# Autodesk Inventor assembly: Test_Assembly
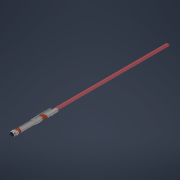
[picture p0: Inventor's stored thumbnail of the model, 180x180]
Saved by Autodesk Inventor 2022 (Build 260153000, 153)
## iProperties
Created: 2024-05-08
Part Number: Test_Assembly
Document SubType Name: Assembly
Designer: jo_ki
Author: jo_ki
## Documents named in this file (16)
- C:\LocalRepos\Lightsaber Git\CAD\LightSaber_Inventor_Project\Assemblies\Blade_Assembly.iam
- C:\LocalRepos\Lightsaber Git\CAD\LightSaber_Inventor_Project\Parts\Blade_Guard.ipt
- C:\LocalRepos\Lightsaber Git\CAD\LightSaber_Inventor_Project\Parts\Saber_Body.ipt
- C:\LocalRepos\Lightsaber Git\CAD\LightSaber_Inventor_Project\Parts\Emitter_Barrel.ipt
- C:\LocalRepos\Lightsaber Git\CAD\LightSaber_Inventor_Project\Parts\Radiator.ipt
- C:\LocalRepos\Lightsaber Git\CAD\LightSaber_Inventor_Project\Parts\Blade.ipt
- C:\LocalRepos\Lightsaber Git\CAD\LightSaber_Inventor_Project\Parts\Endcap.ipt
- C:\LocalRepos\Lightsaber Git\CAD\LightSaber_Inventor_Project\Parts\Decal_Ring_Tripple.ipt
- C:\Users\jo_ki\OneDrive\Dokumente\Inventor\Content Center Files\R2022\en-US\ISO 4762(2)\ISO 4762 - M2.5 x 5ISO.ipt
- C:\Users\jo_ki\OneDrive\Dokumente\Inventor\Content Center Files\R2022\en-US\ISO 4762(2)\ISO 4762 - M2.5 x 4ISO.ipt
- C:\LocalRepos\Lightsaber Git\CAD\LightSaber_Inventor_Project\Parts\Blade_Holder.ipt
- C:\Users\jo_ki\OneDrive\Dokumente\Inventor\Content Center Files\R2022\en-US\DIN 913\DIN 913 - M2.5 x 6.ipt
- C:\Users\jo_ki\OneDrive\Dokumente\Inventor\Content Center Files\R2022\en-US\ISO 4762(2)\ISO 4762 - M2.5 x 10ISO.ipt
- C:\LocalRepos\Lightsaber Git\CAD\LightSaber_Inventor_Project\Assemblies\Electronics_Assembly.iam
- C:\LocalRepos\Lightsaber Git\CAD\LightSaber_Inventor_Project\Parts\Radiator_Disc.ipt
- C:\LocalRepos\Lightsaber Git\CAD\LightSaber_Inventor_Project\Assemblies\Switch_Assembly.iam
## Components (30 placed, 15 different names)
1. Test_Blade_Guard:1 — Mate:1, Mate:52, Insert:2
2. Test_Body:1 — Mate:1, Mate:2, Mate:6, Angle:1, Mate:9, Mate:18, Mate:19, Mate:24, Mate:25, Mate:29, Mate:30, Mate:31, Mate:32, Mate:50, Mate:58, Mate:59, Mate:62, Mate:63, Mate:66, Mate:67, Mate:68, Flush:9, Mate:94
3. Test_Radiator:1 — Mate:9, Mate:50, Mate:51, Mate:54, Mate:71, Mate:72, Mate:73, Mate:74, Mate:75, Mate:76, Mate:77, Mate:78, Mate:79, Mate:80, Mate:81, Mate:82, Mate:83, Mate:84, Mate:85, Mate:86, Mate:89
4. Emitter_Barrel:1 — Mate:2, Mate:51, Mate:52, Mate:56, Mate:57, Mate:60, Mate:61, Insert:3, Insert:4
5. Blade:1 — Mate:19, Flush:1
6. Test_Endcap:1 — Mate:18, Mate:88
7. Test_Decal_Ring_Tripple:1 — Mate:24, Insert:1
8. Test_Decal_Ring_Tripple:2 — Mate:25, Mate:35, Mate:39, Mate:40
9. Test_Blade_Holder:1 — Mate:54, Flush:1
10. Electronics_Assembly:1 [sub-assembly] — Mate:68, Mate:88, Mate:89, Mate:94
11. Test_Radiator_Disc:1 — Mate:74, Mate:79, Flush:2
12. Test_Radiator_Disc:2 — Mate:75, Mate:84, Flush:7, Flush:8
13. Test_Radiator_Disc:3 — Mate:76, Mate:81, Flush:3, Flush:4
14. Test_Radiator_Disc:4 — Mate:77, Mate:82, Flush:4, Flush:5
15. Test_Radiator_Disc:5 — Mate:78, Mate:80, Flush:2, Flush:3
16. Test_Radiator_Disc:6 — Mate:73, Mate:83, Flush:5, Flush:6, Flush:9
17. Test_Radiator_Disc:7 — Mate:72, Flush:6, Flush:7, Mate:86
18. Test_Radiator_Disc:8 — Mate:71, Mate:85, Flush:8
19. Test_Switch_Assembly:1 [sub-assembly]
20. ISO 4762 M2.5 x 5:1 — Mate:29, Mate:30
21. ISO 4762 M2.5 x 5:2 — Mate:31, Mate:32
22. ISO 4762 M2.5 x 4:1 — Mate:39, Mate:40, Mate:67
23. ISO 4762 M2.5 x 4:2 — Insert:1, Mate:66
24. DIN 913 M2.5 x 6:1 — Mate:56, Mate:58
25. DIN 913 M2.5 x 6:2 — Mate:57, Mate:59
26. DIN 913 M2.5 x 6:3 — Mate:60, Mate:63
27. DIN 913 M2.5 x 6:4 — Mate:61, Mate:62
28. ISO 4762 M2.5 x 10:1 — Insert:2
29. ISO 4762 M2.5 x 5:3 — Insert:3
30. ISO 4762 M2.5 x 5:4 — Insert:4
## Relationships (65: Mate 51, Flush 9, Insert 4, Angle 1)
- Mate:1: Test_Blade_Guard:1 ↔ Test_Body:1
- Mate:2: Test_Body:1 ↔ Emitter_Barrel:1
- Mate:6: Test_Body:1
- Angle:1 (0 deg): Test_Body:1
- Mate:9: Test_Body:1 ↔ Test_Radiator:1
- Mate:18: Test_Body:1 ↔ Test_Endcap:1
- Mate:19: Test_Body:1 ↔ Blade:1
- Mate:24: Test_Body:1 ↔ Test_Decal_Ring_Tripple:1
- Mate:25: Test_Body:1 ↔ Test_Decal_Ring_Tripple:2
- Mate:29: Test_Body:1 ↔ ISO 4762 M2.5 x 5:1
- Mate:30: Test_Body:1 ↔ ISO 4762 M2.5 x 5:1
- Mate:31: Test_Body:1 ↔ ISO 4762 M2.5 x 5:2
- Mate:32: Test_Body:1 ↔ ISO 4762 M2.5 x 5:2
- Mate:35: Test_Decal_Ring_Tripple:2
- Mate:37
- Mate:38
- Mate:39: Test_Decal_Ring_Tripple:2 ↔ ISO 4762 M2.5 x 4:1
- Mate:40: Test_Decal_Ring_Tripple:2 ↔ ISO 4762 M2.5 x 4:1
- Insert:1: Test_Decal_Ring_Tripple:1 ↔ ISO 4762 M2.5 x 4:2
- Mate:50: Test_Body:1 ↔ Test_Radiator:1
- Mate:51: Test_Radiator:1 ↔ Emitter_Barrel:1
- Mate:52: Test_Blade_Guard:1 ↔ Emitter_Barrel:1
- Mate:54: Test_Radiator:1 ↔ Test_Blade_Holder:1
- Flush:1: Blade:1 ↔ Test_Blade_Holder:1
- Mate:56: Emitter_Barrel:1 ↔ DIN 913 M2.5 x 6:1
- Mate:57: Emitter_Barrel:1 ↔ DIN 913 M2.5 x 6:2
- Mate:58 (14.25 mm): Test_Body:1 ↔ DIN 913 M2.5 x 6:1
- Mate:59 (14.25 mm): Test_Body:1 ↔ DIN 913 M2.5 x 6:2
- Mate:60: Emitter_Barrel:1 ↔ DIN 913 M2.5 x 6:3
- Mate:61: Emitter_Barrel:1 ↔ DIN 913 M2.5 x 6:4
- Mate:62 (14.25 mm): Test_Body:1 ↔ DIN 913 M2.5 x 6:4
- Mate:63 (14.25 mm): Test_Body:1 ↔ DIN 913 M2.5 x 6:3
- Insert:2: Test_Blade_Guard:1 ↔ ISO 4762 M2.5 x 10:1
- Insert:3: Emitter_Barrel:1 ↔ ISO 4762 M2.5 x 5:3
- Insert:4: Emitter_Barrel:1 ↔ ISO 4762 M2.5 x 5:4
- Mate:66: Test_Body:1 ↔ ISO 4762 M2.5 x 4:2
- Mate:67: Test_Body:1 ↔ ISO 4762 M2.5 x 4:1
- Mate:68: Test_Body:1 ↔ Electronics_Assembly:1
- Mate:71: Test_Radiator:1 ↔ Test_Radiator_Disc:8
- Mate:72: Test_Radiator:1 ↔ Test_Radiator_Disc:7
- Mate:73: Test_Radiator:1 ↔ Test_Radiator_Disc:6
- Mate:74: Test_Radiator:1 ↔ Test_Radiator_Disc:1
- Mate:75: Test_Radiator:1 ↔ Test_Radiator_Disc:2
- Mate:76: Test_Radiator:1 ↔ Test_Radiator_Disc:3
- Mate:77: Test_Radiator:1 ↔ Test_Radiator_Disc:4
- Mate:78: Test_Radiator:1 ↔ Test_Radiator_Disc:5
- Mate:79: Test_Radiator:1 ↔ Test_Radiator_Disc:1
- Mate:80: Test_Radiator:1 ↔ Test_Radiator_Disc:5
- Mate:81: Test_Radiator:1 ↔ Test_Radiator_Disc:3
- Mate:82: Test_Radiator:1 ↔ Test_Radiator_Disc:4
- Mate:83: Test_Radiator:1 ↔ Test_Radiator_Disc:6
- Mate:84: Test_Radiator:1 ↔ Test_Radiator_Disc:2
- Mate:85: Test_Radiator:1 ↔ Test_Radiator_Disc:8
- Flush:2: Test_Radiator_Disc:1 ↔ Test_Radiator_Disc:5
- Flush:3: Test_Radiator_Disc:3 ↔ Test_Radiator_Disc:5
- Flush:4: Test_Radiator_Disc:3 ↔ Test_Radiator_Disc:4
- Flush:5: Test_Radiator_Disc:4 ↔ Test_Radiator_Disc:6
- Flush:6: Test_Radiator_Disc:6 ↔ Test_Radiator_Disc:7
- Flush:7: Test_Radiator_Disc:2 ↔ Test_Radiator_Disc:7
- Flush:8: Test_Radiator_Disc:2 ↔ Test_Radiator_Disc:8
- Flush:9: Test_Body:1 ↔ Test_Radiator_Disc:6
- Mate:86: Test_Radiator:1 ↔ Test_Radiator_Disc:7
- Mate:88: Test_Endcap:1 ↔ Electronics_Assembly:1
- Mate:89: Test_Radiator:1 ↔ Electronics_Assembly:1
- Mate:94: Test_Body:1 ↔ Electronics_Assembly:1
